# Autodesk Inventor assembly: LiDAR
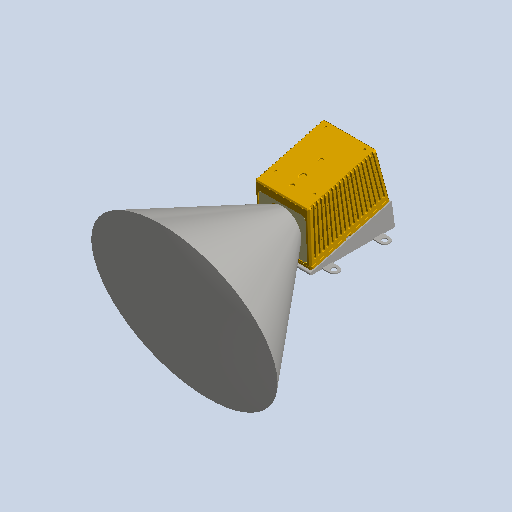
[picture p0: Inventor's stored thumbnail of the model, 512x512]
Saved by Autodesk Inventor 2022.1 (Build 261234000, 234)
## iProperties
Part Number: LiDAR
Document SubType Name: Ensamblaje
Designer: seb_0
Author: seb_0
## Documents named in this file (3)
- C:\Users\seb_0\Desktop\PDM\ProyectoRobotPallet\LiDAR\LiDAR.iam
- C:\Users\seb_0\Desktop\PDM\ProyectoRobotPallet\LiDAR\Soporte_LíDAR.ipt
- C:\Users\seb_0\Desktop\PDM\ProyectoRobotPallet\LiDAR\Livox Mid-70.ipt
## Components (2 placed, 2 different names)
1. Soporte_LíDAR:1 — Coincidencia:1, Coincidencia:2, Coincidencia:3, Coincidencia:4, Coincidencia:5
2. Livox Mid-70:1 — Coincidencia:3, Coincidencia:4, Coincidencia:5
## Relationships (5: Mate 5)
- Coincidencia:1 [Mate]: Soporte_LíDAR:1
- Coincidencia:2 [Mate]: Soporte_LíDAR:1
- Coincidencia:3 [Mate]: Soporte_LíDAR:1 ↔ Livox Mid-70:1
- Coincidencia:4 [Mate]: Soporte_LíDAR:1 ↔ Livox Mid-70:1
- Coincidencia:5 [Mate]: Soporte_LíDAR:1 ↔ Livox Mid-70:1
